# Autodesk Inventor assembly: WCP-0416 - GreyT Telescope Gearbox (Stages #1-4)_2" - Base Gearbox
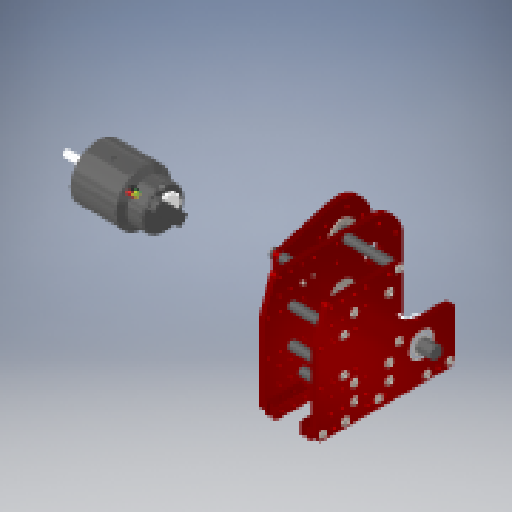
[picture p0: Inventor's stored thumbnail of the model, 512x512]
Saved by Autodesk Inventor 2024.2 (Build 282272000, 272)
## iProperties
Created: 2024-01-30
Part Number: WCP-0416 - GreyT Telescope Gearbox (Stages #1-4)_2" - Base Gearbox
Document SubType Name: Assembly
Designer: rohan
Author: rohan
Revision Number: ANY
## Documents named in this file (33)
- C:\Users\rohan\OneDrive - Hillsborough County Public Schools\Robotics\FIRST-Robotics-Competition\Crescendo\Minotaur-Crescendo-Robot\Structure\Superstructure\Climber\WCP - Greyt Telescope (Stages 1-4)\WCP-0416 -_1.iam
- C:\Users\rohan\OneDrive - Hillsborough County Public Schools\Robotics\FIRST-Robotics-Competition\Crescendo\Minotaur-Crescendo-Robot\Structure\Superstructure\Climber\WCP - Greyt Telescope (Stages 1-4)\WCP-0416-0.ipt
- C:\Users\rohan\OneDrive - Hillsborough County Public Schools\Robotics\FIRST-Robotics-Competition\Crescendo\Minotaur-Crescendo-Robot\Structure\Superstructure\Climber\WCP - Greyt Telescope (Stages 1-4)\WCP-0416-0_1.ipt
- C:\Users\rohan\OneDrive - Hillsborough County Public Schools\Robotics\FIRST-Robotics-Competition\Crescendo\Minotaur-Crescendo-Robot\Structure\Superstructure\Climber\WCP - Greyt Telescope (Stages 1-4)\WCP-0416-0_2.ipt
- C:\Users\rohan\OneDrive - Hillsborough County Public Schools\Robotics\FIRST-Robotics-Competition\Crescendo\Minotaur-Crescendo-Robot\Structure\Superstructure\Climber\WCP - Greyt Telescope (Stages 1-4)\WCP-0225-0.ipt
- C:\Users\rohan\OneDrive - Hillsborough County Public Schools\Robotics\FIRST-Robotics-Competition\Crescendo\Minotaur-Crescendo-Robot\Structure\Superstructure\Climber\WCP - Greyt Telescope (Stages 1-4)\WCP-0416-0_7.ipt
- C:\Users\rohan\OneDrive - Hillsborough County Public Schools\Robotics\FIRST-Robotics-Competition\Crescendo\Minotaur-Crescendo-Robot\Structure\Superstructure\Climber\WCP - Greyt Telescope (Stages 1-4)\WCP-0443 R.ipt
- C:\Users\rohan\OneDrive - Hillsborough County Public Schools\Robotics\FIRST-Robotics-Competition\Crescendo\Minotaur-Crescendo-Robot\Structure\Superstructure\Climber\WCP - Greyt Telescope (Stages 1-4)\Falcon_Mot.ipt
- C:\Users\rohan\OneDrive - Hillsborough County Public Schools\Robotics\FIRST-Robotics-Competition\Crescendo\Minotaur-Crescendo-Robot\Structure\Superstructure\Climber\WCP - Greyt Telescope (Stages 1-4)\217-2731_0.ipt
- C:\Users\rohan\OneDrive - Hillsborough County Public Schools\Robotics\FIRST-Robotics-Competition\Crescendo\Minotaur-Crescendo-Robot\Structure\Superstructure\Climber\WCP - Greyt Telescope (Stages 1-4)\217-4006_0.ipt
- C:\Users\rohan\OneDrive - Hillsborough County Public Schools\Robotics\FIRST-Robotics-Competition\Crescendo\Minotaur-Crescendo-Robot\Structure\Superstructure\Climber\WCP - Greyt Telescope (Stages 1-4)\217-3875_0.ipt
- C:\Users\rohan\OneDrive - Hillsborough County Public Schools\Robotics\FIRST-Robotics-Competition\Crescendo\Minotaur-Crescendo-Robot\Structure\Superstructure\Climber\WCP - Greyt Telescope (Stages 1-4)\217-3573_5.ipt
- C:\Users\rohan\OneDrive - Hillsborough County Public Schools\Robotics\FIRST-Robotics-Competition\Crescendo\Minotaur-Crescendo-Robot\Structure\Superstructure\Climber\WCP - Greyt Telescope (Stages 1-4)\217-3209_1.ipt
- C:\Users\rohan\OneDrive - Hillsborough County Public Schools\Robotics\FIRST-Robotics-Competition\Crescendo\Minotaur-Crescendo-Robot\Structure\Superstructure\Climber\WCP - Greyt Telescope (Stages 1-4)\WCP-0226 R.ipt
- C:\Users\rohan\OneDrive - Hillsborough County Public Schools\Robotics\FIRST-Robotics-Competition\Crescendo\Minotaur-Crescendo-Robot\Structure\Superstructure\Climber\WCP - Greyt Telescope (Stages 1-4)\WCP-0207 R.ipt
- C:\Users\rohan\OneDrive - Hillsborough County Public Schools\Robotics\FIRST-Robotics-Competition\Crescendo\Minotaur-Crescendo-Robot\Structure\Superstructure\Climber\WCP - Greyt Telescope (Stages 1-4)\WCP-0307 R.ipt
- C:\Users\rohan\OneDrive - Hillsborough County Public Schools\Robotics\FIRST-Robotics-Competition\Crescendo\Minotaur-Crescendo-Robot\Structure\Superstructure\Climber\WCP - Greyt Telescope (Stages 1-4)\10-32 BHCS_5.ipt
- C:\Users\rohan\OneDrive - Hillsborough County Public Schools\Robotics\FIRST-Robotics-Competition\Crescendo\Minotaur-Crescendo-Robot\Structure\Superstructure\Climber\WCP - Greyt Telescope (Stages 1-4)\10-32 BHCS_2.ipt
- C:\Users\rohan\OneDrive - Hillsborough County Public Schools\Robotics\FIRST-Robotics-Competition\Crescendo\Minotaur-Crescendo-Robot\Structure\Superstructure\Climber\WCP - Greyt Telescope (Stages 1-4)\10-32 BHCS_1.ipt
- C:\Users\rohan\OneDrive - Hillsborough County Public Schools\Robotics\FIRST-Robotics-Competition\Crescendo\Minotaur-Crescendo-Robot\Structure\Superstructure\Climber\WCP - Greyt Telescope (Stages 1-4)\10-32 BHCS_6.ipt
- C:\Users\rohan\OneDrive - Hillsborough County Public Schools\Robotics\FIRST-Robotics-Competition\Crescendo\Minotaur-Crescendo-Robot\Structure\Superstructure\Climber\WCP - Greyt Telescope (Stages 1-4)\10-32 BHCS_3.ipt
- C:\Users\rohan\OneDrive - Hillsborough County Public Schools\Robotics\FIRST-Robotics-Competition\Crescendo\Minotaur-Crescendo-Robot\Structure\Superstructure\Climber\WCP - Greyt Telescope (Stages 1-4)\217-3259_2.ipt
- C:\Users\rohan\OneDrive - Hillsborough County Public Schools\Robotics\FIRST-Robotics-Competition\Crescendo\Minotaur-Crescendo-Robot\Structure\Superstructure\Climber\WCP - Greyt Telescope (Stages 1-4)\217-3257_0.ipt
- C:\Users\rohan\OneDrive - Hillsborough County Public Schools\Robotics\FIRST-Robotics-Competition\Crescendo\Minotaur-Crescendo-Robot\Structure\Superstructure\Climber\WCP - Greyt Telescope (Stages 1-4)\WCP-0189 R.ipt
- C:\Users\rohan\OneDrive - Hillsborough County Public Schools\Robotics\FIRST-Robotics-Competition\Crescendo\Minotaur-Crescendo-Robot\Structure\Superstructure\Climber\WCP - Greyt Telescope (Stages 1-4)\217-3283 R.ipt
- C:\Users\rohan\OneDrive - Hillsborough County Public Schools\Robotics\FIRST-Robotics-Competition\Crescendo\Minotaur-Crescendo-Robot\Structure\Superstructure\Climber\WCP - Greyt Telescope (Stages 1-4)\WCP-0282 R.ipt
- C:\Users\rohan\OneDrive - Hillsborough County Public Schools\Robotics\FIRST-Robotics-Competition\Crescendo\Minotaur-Crescendo-Robot\Structure\Superstructure\Climber\WCP - Greyt Telescope (Stages 1-4)\WCP-0416-0_4.ipt
- C:\Users\rohan\OneDrive - Hillsborough County Public Schools\Robotics\FIRST-Robotics-Competition\Crescendo\Minotaur-Crescendo-Robot\Structure\Superstructure\Climber\WCP - Greyt Telescope (Stages 1-4)\WCP-0229 R.ipt
- C:\Users\rohan\OneDrive - Hillsborough County Public Schools\Robotics\FIRST-Robotics-Competition\Crescendo\Minotaur-Crescendo-Robot\Structure\Superstructure\Climber\WCP - Greyt Telescope (Stages 1-4)\WCP-0416-0_5.ipt
- C:\Users\rohan\OneDrive - Hillsborough County Public Schools\Robotics\FIRST-Robotics-Competition\Crescendo\Minotaur-Crescendo-Robot\Structure\Superstructure\Climber\WCP - Greyt Telescope (Stages 1-4)\WCP-0416-0_6.ipt
- C:\Users\rohan\OneDrive - Hillsborough County Public Schools\Robotics\FIRST-Robotics-Competition\Crescendo\Minotaur-Crescendo-Robot\Structure\Superstructure\Climber\WCP - Greyt Telescope (Stages 1-4)\CANcoder.ipt
- C:\Users\rohan\OneDrive - Hillsborough County Public Schools\Robotics\FIRST-Robotics-Competition\Crescendo\Minotaur-Crescendo-Robot\Structure\Superstructure\Climber\WCP - Greyt Telescope (Stages 1-4)\WCP-0156 R.ipt
- C:\Users\rohan\OneDrive - Hillsborough County Public Schools\Robotics\FIRST-Robotics-Competition\Crescendo\Minotaur-Crescendo-Robot\Electronics\Neo-Brushless-Motors\NEO-Brushless-Motor-V1.0.ipt
## Components (79 placed, 79 different names)
1. WCP-0416-001 Rev1_251
2. WCP-0416-002 Rev1_252
3. WCP-0416-003 Rev1_253
4. WCP-0225-006 Rev1_254
5. WCP-0416-007 Rev1_2" Gearbox_255
6. WCP-0443 Rev1_256
7. WCP-0443 Rev1_257
8. Falcon_Motor_Spacer_0625_259 — Mate:2
9. 217-2731_0_500_flanged_bearing_260
10. 217-2731_0_500_flanged_bearing_261
11. 217-4006_0_500_flanged_thunderhex_bearing_262
12. 217-3875_0_500_flanged_hex_bearing_263
13. 217-2731_0_500_flanged_bearing_264
14. 217-3573_54T_500_hex_265
15. 217-3573_54T_500_hex_266
16. 217-3209_18T_500_hex_267
17. WCP-0226 Rev1_269
18. WCP-0226 Rev1_270
19. WCP-0226 Rev1_271
20. WCP-0226 Rev1_272
21. WCP-0207 Rev1_273
22. WCP-0207 Rev1_274
23. WCP-0207 Rev1_275
24. WCP-0207 Rev1_276
25. WCP-0207 Rev1_277
26. WCP-0307 Rev1_278
27. WCP-0307 Rev1_279
28. WCP-0207 Rev1_280
29. WCP-0207 Rev1_281
30. 10-32 BHCS - No Thread_1.750_282
31. 10-32 BHCS - No Thread_1.750_284
32. 10-32 BHCS - No Thread_1.750_285
33. 10-32 BHCS - No Thread_0.500_286
34. 10-32 BHCS - No Thread_0.500_287
35. 10-32 BHCS - No Thread_0.375_288
36. 10-32 BHCS - No Thread_0.375_289
37. 10-32 BHCS - No Thread_0.375_290
38. 10-32 BHCS - No Thread_0.375_291
39. 10-32 BHCS - No Thread_0.250_292
40. 10-32 BHCS - No Thread_0.375_293
41. 10-32 BHCS - No Thread_2.500_294
42. 10-32 BHCS - No Thread_2.500_295
43. 10-32 BHCS - No Thread_2.500_296
44. 10-32 BHCS - No Thread_2.500_297
45. 10-32 BHCS - No Thread_2.500_298
46. 10-32 BHCS - No Thread_2.500_299
47. 10-32 BHCS - No Thread_0.375_300
48. 10-32 BHCS - No Thread_0.375_301
49. 10-32 BHCS - No Thread_0.250_302
50. 10-32 BHCS - No Thread_0.250_303
51. 10-32 BHCS - No Thread_0.500_304
52. 10-32 BHCS - No Thread_0.500_305
53. 10-32 BHCS - No Thread_0.500_306
54. 10-32 BHCS - No Thread_0.500_307
55. 10-32 BHCS - No Thread_0.500_308
56. 10-32 BHCS - No Thread_0.500_309
57. 10-32 BHCS - No Thread_0.500_310
58. 10-32 BHCS - No Thread_0.500_311
59. 10-32 BHCS - No Thread_0.500_312
60. 10-32 BHCS - No Thread_0.500_313
61. 10-32 BHCS - No Thread_2.500_314
62. 217-3259_250L_500_hex_315 — Mate:1
63. 217-3257_0625L_500_hex_316
64. 217-3257_0625L_500_hex_317
65. WCP-0189 Rev1_318
66. WCP-0189 Rev1_319
67. 217-3283 Rev1_320
68. WCP-0282 Rev1_321
69. WCP-0416-009 Rev1_322
70. WCP-0416-009 Rev1_323
71. WCP-0416-009 Rev1_324
72. WCP-0416-009 Rev1_325
73. WCP-0229 Rev1_326
74. WCP-0229 Rev1_327
75. WCP-0416-008 Rev1_328
76. WCP-0416-010 Rev1_329
77. CANcoder_335
78. WCP-0156 Rev1_336
79. NEO-Brushless-Motor-V1.0:1 — Mate:1, Mate:2
## Relationships (2: Mate 2)
- Mate:1: 217-3259_250L_500_hex_315 ↔ NEO-Brushless-Motor-V1.0:1
- Mate:2: Falcon_Motor_Spacer_0625_259 ↔ NEO-Brushless-Motor-V1.0:1
